# Autodesk Inventor assembly: Truck 2
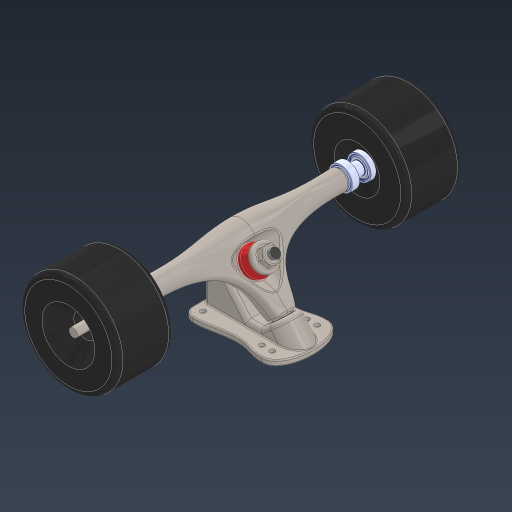
[picture p0: Inventor's stored thumbnail of the model, 512x512]
Saved by Autodesk Inventor 2023 (Build 270158000, 158)
## iProperties
Created: 2025-11-14
Part Number: Truck 2
Document SubType Name: Assembly
Designer: szymo
Author: szymo
Revision Number: ANY
## Documents named in this file (15)
- D:\tech\diy\e-skateboard\projekcik-inventor\longboard\Truck 2.iam
- D:\tech\diy\e-skateboard\projekcik-inventor\longboard\Plato base.ipt
- D:\tech\diy\e-skateboard\projekcik-inventor\longboard\Ala.ipt
- D:\tech\diy\e-skateboard\projekcik-inventor\longboard\Buje grande.ipt
- D:\tech\diy\e-skateboard\projekcik-inventor\longboard\Arandela grande Kingpin.ipt
- D:\tech\diy\e-skateboard\projekcik-inventor\longboard\Buje pequeño.ipt
- D:\tech\diy\e-skateboard\projekcik-inventor\longboard\Arandela pequeña Kingpin.ipt
- D:\tech\diy\e-skateboard\projekcik-inventor\longboard\King Pin.ipt
- D:\tech\diy\e-skateboard\projekcik-inventor\longboard\Tuerca 3_8.ipt
- D:\tech\diy\e-skateboard\projekcik-inventor\longboard\Ball Bearing 608ZZ_Dfaut.ipt
- D:\tech\diy\e-skateboard\projekcik-inventor\longboard\Arandela 8mm.ipt
- D:\tech\diy\e-skateboard\projekcik-inventor\longboard\Rueda.ipt
- D:\tech\diy\e-skateboard\projekcik-inventor\longboard\Buje.ipt
- D:\tech\diy\e-skateboard\projekcik-inventor\longboard\prevailing torque hex nut_am_AM-M8-N.ipt
- D:\tech\diy\e-skateboard\projekcik-inventor\longboard\Buje de Goma.ipt
## Components (23 placed, 23 different names)
1. Plato base_20
2. Ala_21 — Mate:1, Flush:1, Mate:2, Flush:2
3. Buje grande_22
4. Arandela grande Kingpin_23
5. Buje pequeño_24
6. Arandela pequeña Kingpin_25
7. King Pin_26
8. Tuerca 3_8_27
9. Ball Bearing 608ZZ_Dfaut_28
10. Ball Bearing 608ZZ_Dfaut_29
11. Ball Bearing 608ZZ_Dfaut_30
12. Ball Bearing 608ZZ_Dfaut_31
13. Arandela 8mm_32
14. Arandela 8mm_33
15. Arandela 8mm_34
16. Arandela 8mm_35
17. Rueda_36 — Mate:2, Flush:2
18. Rueda_37 — Mate:1, Flush:1
19. Buje_38
20. Buje_39
21. prevailing torque hex nut_am_AM-M8-N_40
22. prevailing torque hex nut_am_AM-M8-N_41
23. Buje de Goma_42
## Relationships (4: Mate 2, Flush 2)
- Mate:1: Ala_21 ↔ Rueda_37
- Flush:1 (-4.5 mm): Ala_21 ↔ Rueda_37
- Mate:2: Ala_21 ↔ Rueda_36
- Flush:2 (-4.5 mm): Ala_21 ↔ Rueda_36
